# Autodesk Inventor assembly: Batt holder sestava
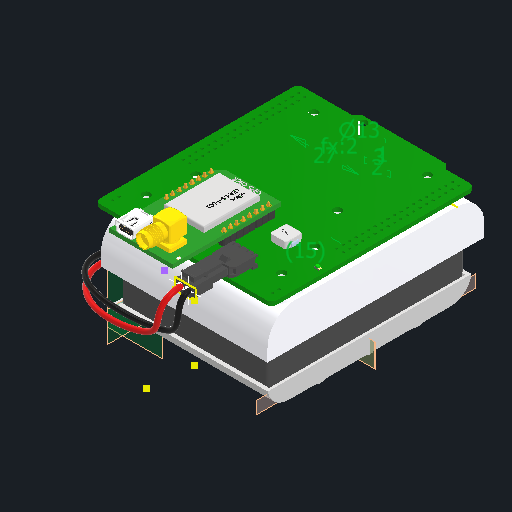
[picture p0: Inventor's stored thumbnail of the model, 512x512]
Saved by Autodesk Inventor 2022 (Build 260153000, 153)
## iProperties
Created: 2022-03-27
Part Number: Batt holder sestava
Document SubType Name: Assembly
Designer: dvorakj
Author: dvorakj
## Documents named in this file (5)
- C:\Users\dvorakj\Documents\Inventor\Bakalarka\Batt holder\Batt holder sestava.iam
- C:\Users\dvorakj\Documents\Inventor\Bakalarka\Batt holder\Batt_holder.ipt
- C:\Users\dvorakj\Documents\Inventor\Bakalarka\altium export\Shield_bot\shield_bot_sestava.iam
- C:\Users\dvorakj\Documents\Inventor\Bakalarka\Batt_holder_holder\batt holder holder.ipt
- C:\Users\dvorakj\Documents\Inventor\Bakalarka\Batt_holder_holder_bot\Batt holder holder_bot.ipt
## Components (4 placed, 4 different names)
1. Batt_holder:1 — Angle:1, Mate:2, Angle:2, Flush:2, Flush:3, Mate:11, Mate:12, Mate:13
2. shield_bot_sestava:1 [sub-assembly] — Mate:11
3. batt holder holder:1 — Flush:2, Flush:3, Angle:3
4. Batt holder holder_bot:1 — Mate:12, Mate:13, Angle:3
## Relationships (12: Mate 4, Angle 3, Flush 3, Symmetry 2)
- Angle:1 (0 deg): Batt_holder:1
- Mate:2: Batt_holder:1
- Angle:2 (0 deg): Batt_holder:1
- Symmetry:1
- Symmetry:2
- Flush:1
- Flush:2: Batt_holder:1 ↔ batt holder holder:1
- Flush:3: Batt_holder:1 ↔ batt holder holder:1
- Mate:11: Batt_holder:1 ↔ shield_bot_sestava:1
- Mate:12: Batt_holder:1 ↔ Batt holder holder_bot:1
- Mate:13 (0.5 mm): Batt_holder:1 ↔ Batt holder holder_bot:1
- Angle:3 (180 deg): batt holder holder:1 ↔ Batt holder holder_bot:1
